# Autodesk Inventor assembly: SAR330 + fixed couplers left
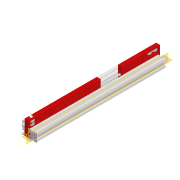
[picture p0: Inventor's stored thumbnail of the model, 180x180]
Saved by Autodesk Inventor 2020 (Build 240168000, 168)
## iProperties
Created: 2019-11-17
Part Number: SAR330 + fixed couplers left
Document SubType Name: Assembly
Designer: ball
Author: ball
## Documents named in this file (8)
- C:\FTC\FTC8863CAD\2019 Robot\Delivery\SAR330 + fixed couplers left.iam
- C:\FTC\FTC8863CAD\Misumi\SAR330\SAR330 440 offset.iam
- C:\FTC\FTC8863CAD\Actobotics\634 parts\634266.ipt
- C:\FTC\FTC8863CAD\StepLibraries\Screws\M3 x 20 HEX HEAD CAP SCREW.ipt
- C:\FTC\FTC8863CAD\Actobotics\565 parts\565046.ipt
- C:\FTC\FTC8863CAD\StepLibraries\Screws\6-32x.375_18-8 SS TRUSS HEAD PHILLIPS MACHINE SCREW.ipt
- C:\FTC\FTC8863CAD\2019 Robot\Delivery\Coupler lift short top left + pulleys.iam
- C:\FTC\FTC8863CAD\2019 Robot\Delivery\Coupler lift long bottom left + pulleys.iam
## Components (7 placed, 7 different names)
1. SAR330 440 offset:1 [sub-assembly] — Mate:3, Mate:4, Angle:2, Mate:5, Mate:6, Mate:7
2. Coupler lift short top left + pulleys:1 [sub-assembly] — Mate:3, Mate:4, Angle:2
3. 634266:1
4. Coupler lift long bottom left + pulleys:1 [sub-assembly] — Mate:5, Mate:6, Mate:7, Mate:8, Mate:9, Mate:10, Flush:1, Flush:2, Mate:11, Mate:12
5. M3 x 20 HEX HEAD CAP SCREW:1 — Mate:8, Mate:9
6. 565046:1 — Mate:10, Flush:1, Flush:2
7. 6-32x.375_18-8 SS TRUSS HEAD PHILLIPS MACHINE SCREW:1 — Mate:11, Mate:12
## Relationships (13: Mate 10, Flush 2, Angle 1)
- Mate:3: SAR330 440 offset:1 ↔ Coupler lift short top left + pulleys:1
- Mate:4: SAR330 440 offset:1 ↔ Coupler lift short top left + pulleys:1
- Angle:2 (0 deg): SAR330 440 offset:1 ↔ Coupler lift short top left + pulleys:1
- Mate:5: SAR330 440 offset:1 ↔ Coupler lift long bottom left + pulleys:1
- Mate:6: SAR330 440 offset:1 ↔ Coupler lift long bottom left + pulleys:1
- Mate:7: SAR330 440 offset:1 ↔ Coupler lift long bottom left + pulleys:1
- Mate:8: Coupler lift long bottom left + pulleys:1 ↔ M3 x 20 HEX HEAD CAP SCREW:1
- Mate:9: Coupler lift long bottom left + pulleys:1 ↔ M3 x 20 HEX HEAD CAP SCREW:1
- Mate:10: Coupler lift long bottom left + pulleys:1 ↔ 565046:1
- Flush:1: Coupler lift long bottom left + pulleys:1 ↔ 565046:1
- Flush:2: Coupler lift long bottom left + pulleys:1 ↔ 565046:1
- Mate:11: Coupler lift long bottom left + pulleys:1 ↔ 6-32x.375_18-8 SS TRUSS HEAD PHILLIPS MACHINE SCREW:1
- Mate:12: Coupler lift long bottom left + pulleys:1 ↔ 6-32x.375_18-8 SS TRUSS HEAD PHILLIPS MACHINE SCREW:1
